# Autodesk Inventor assembly: Assembly
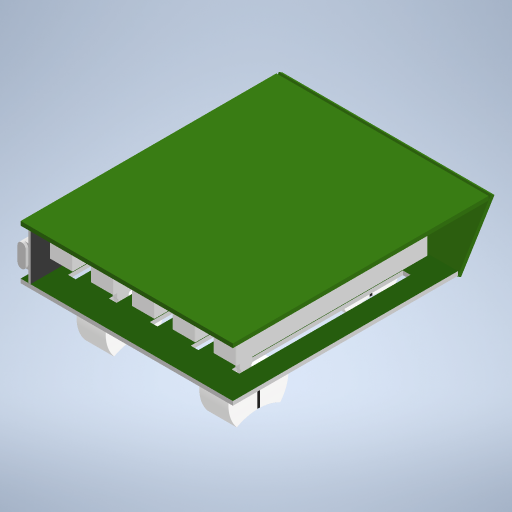
[picture p0: Inventor's stored thumbnail of the model, 512x512]
Saved by Autodesk Inventor 2023 (Build 270158000, 158)
## iProperties
Created: 2024-03-19
Part Number: Assembly
Document SubType Name: Assembly
Designer: noname
Author: noname
## Documents named in this file (7)
- C:\Users\noname\Documents\GitHub\AudMix\3dModels\Assembly.iam
- C:\Users\noname\Documents\GitHub\AudMix\3dModels\Slider\SliderAssembly.iam
- C:\Users\noname\Documents\GitHub\AudMix\3dModels\TopPCB.ipt
- C:\Users\noname\Documents\GitHub\AudMix\3dModels\Part7.ipt
- C:\Users\noname\Documents\GitHub\AudMix\3dModels\Part8.ipt
- C:\Users\noname\Documents\GitHub\AudMix\3dModels\0_42_oled.ipt
- C:\Users\noname\Documents\GitHub\AudMix\3dModels\rp2040.ipt
## Components (14 placed, 6 different names)
1. SliderAssembly:1 [sub-assembly] — Mate:1, Mate:2, Flush:1, Flush:2, Flush:3, Flush:7, Flush:10, Flush:21
2. TopPCB:1 — Mate:1, Mate:2, Flush:1, Flush:4, Flush:11, Flush:12, Flush:13, Flush:14
3. SliderAssembly:2 [sub-assembly] — Flush:2, Flush:3, Flush:4, Flush:5, Flush:6, Flush:8, Flush:20
4. SliderAssembly:3 [sub-assembly] — Flush:5, Flush:8, Flush:9, Flush:11, Flush:19
5. SliderAssembly:4 [sub-assembly] — Flush:6, Flush:9, Flush:12, Flush:18
6. SliderAssembly:5 [sub-assembly] — Flush:7, Flush:10, Flush:13, Flush:17
7. Part7:1 — Flush:15, Flush:16, Flush:26, Mate:8
8. Part8:1 — Flush:16, Mate:3, Mate:4, Mate:5, Mate:6, Mate:7
9. 0_42_oled:1 — Mate:3, Flush:17, Flush:22
10. 0_42_oled:2 — Mate:4, Flush:18, Flush:22, Flush:23
11. 0_42_oled:3 — Mate:5, Flush:19, Flush:23, Flush:24
12. 0_42_oled:4 — Mate:6, Flush:20, Flush:24, Flush:25
13. 0_42_oled:5 — Mate:7, Flush:21, Flush:25
14. rp2040:1 — Flush:26, Mate:8
## Relationships (34: Flush 26, Mate 8)
- Mate:1 (6 mm): SliderAssembly:1 ↔ TopPCB:1
- Mate:2 (0.5 mm): SliderAssembly:1 ↔ TopPCB:1
- Flush:1: SliderAssembly:1 ↔ TopPCB:1
- Flush:2: SliderAssembly:1 ↔ SliderAssembly:2
- Flush:3: SliderAssembly:1 ↔ SliderAssembly:2
- Flush:4 (0.5 mm): TopPCB:1 ↔ SliderAssembly:2
- Flush:5: SliderAssembly:2 ↔ SliderAssembly:3
- Flush:6: SliderAssembly:2 ↔ SliderAssembly:4
- Flush:7: SliderAssembly:1 ↔ SliderAssembly:5
- Flush:8: SliderAssembly:2 ↔ SliderAssembly:3
- Flush:9: SliderAssembly:3 ↔ SliderAssembly:4
- Flush:10: SliderAssembly:1 ↔ SliderAssembly:5
- Flush:11 (-0.5 mm): TopPCB:1 ↔ SliderAssembly:3
- Flush:12 (-0.5 mm): TopPCB:1 ↔ SliderAssembly:4
- Flush:13 (-0.5 mm): TopPCB:1 ↔ SliderAssembly:5
- Flush:14 (17.9 mm): TopPCB:1
- Flush:15: Part7:1
- Flush:16: Part7:1 ↔ Part8:1
- Mate:3: Part8:1 ↔ 0_42_oled:1
- Flush:17 (-1.5 mm): SliderAssembly:5 ↔ 0_42_oled:1
- Mate:4: Part8:1 ↔ 0_42_oled:2
- Mate:5: Part8:1 ↔ 0_42_oled:3
- Mate:6: Part8:1 ↔ 0_42_oled:4
- Mate:7: Part8:1 ↔ 0_42_oled:5
- Flush:18 (-1.5 mm): SliderAssembly:4 ↔ 0_42_oled:2
- Flush:19 (-1.5 mm): SliderAssembly:3 ↔ 0_42_oled:3
- Flush:20 (-1.5 mm): SliderAssembly:2 ↔ 0_42_oled:4
- Flush:21 (-1.5 mm): SliderAssembly:1 ↔ 0_42_oled:5
- Flush:22: 0_42_oled:1 ↔ 0_42_oled:2
- Flush:23: 0_42_oled:2 ↔ 0_42_oled:3
- Flush:24: 0_42_oled:3 ↔ 0_42_oled:4
- Flush:25: 0_42_oled:4 ↔ 0_42_oled:5
- Flush:26 (3 mm): Part7:1 ↔ rp2040:1
- Mate:8: Part7:1 ↔ rp2040:1
